# Autodesk Inventor assembly: A02_R01 - Main Shaft Assembly
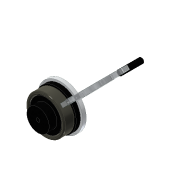
[picture p0: Inventor's stored thumbnail of the model, 180x180]
Saved by Autodesk Inventor 2016 (Build 200138000, 138)
## iProperties
Created: 2017-02-27
Part Number: A02_R01 - Main Shaft Assembly
Document SubType Name: Conjunto soldado
Designer: Fernando
Weld Material: Aço macio soldado
Mass: 1898.58 g
Surface Area: 1056.77 cm^2
Volume: 365.841 cm^3
Density: 5.18962 g/cm^3
SurfaceArea_m2: .11
Author: Fernando
## Documents named in this file (7)
- G:\00 - Files\00 - Personal\40 - Hobbies\90 - Projetos Particulares\40 - POV Display\01 - Mechanical Design\A02_R01 - Main Shaft Assembly.iam
- G:\00 - Files\00 - Personal\40 - Hobbies\90 - Projetos Particulares\40 - POV Display\01 - Mechanical Design\M17 - Coil Support Part.ipt
- G:\00 - Files\00 - Personal\40 - Hobbies\90 - Projetos Particulares\40 - POV Display\01 - Mechanical Design\P04 - M8 Left Nut.ipt
- G:\00 - Files\00 - Personal\40 - Hobbies\90 - Projetos Particulares\40 - POV Display\01 - Mechanical Design\M16 - RX Coil.ipt
- G:\00 - Files\00 - Personal\40 - Hobbies\90 - Projetos Particulares\40 - POV Display\01 - Mechanical Design\M02_R01 - Main Spherical Shaft.ipt
- G:\00 - Files\00 - Personal\40 - Hobbies\90 - Projetos Particulares\40 - POV Display\01 - Mechanical Design\M19 - Dowel.ipt
- G:\00 - Files\00 - Personal\40 - Hobbies\90 - Projetos Particulares\40 - POV Display\01 - Mechanical Design\M20 - Flange Connector.ipt
## Components (6 placed, 6 different names)
1. M17 - Coil Support Part:1 — Insert:1, Insert:2, Insert:3, Mate:13
2. P04 - M8 Left Nut:1 — Insert:1
3. M16 - RX Coil:1 — Insert:2
4. M02_R01 - Main Spherical Shaft:1 — Insert:4, Mate:14
5. M19 - Dowel:1 — Mate:11
6. M20 - Flange Connector:1 — Insert:3, Mate:13, Insert:4, Mate:14
## Relationships (7: Insert 4, Mate 3)
- Insert:1: M17 - Coil Support Part:1 ↔ P04 - M8 Left Nut:1
- Insert:2: M17 - Coil Support Part:1 ↔ M16 - RX Coil:1
- Mate:11: M19 - Dowel:1
- Insert:3: M17 - Coil Support Part:1 ↔ M20 - Flange Connector:1
- Mate:13: M17 - Coil Support Part:1 ↔ M20 - Flange Connector:1
- Insert:4: M02_R01 - Main Spherical Shaft:1 ↔ M20 - Flange Connector:1
- Mate:14 (0.1 mm): M02_R01 - Main Spherical Shaft:1 ↔ M20 - Flange Connector:1
